(part 1 of 2)
# Autodesk Inventor assembly: Drive Roller Assembly 2
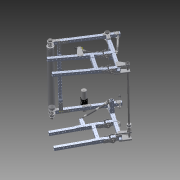
[picture p0: Inventor's stored thumbnail of the model, 180x180]
Saved by Autodesk Inventor 2014 SP1 (Build 180222100, 222)
## iProperties
Created: 2014-01-12
Part Number: Drive Roller Assembly 2
Document SubType Name: Assembly
Designer: Michael
Mass: 6489.5 g
Surface Area: 18387.5 cm^2
Volume: 1765.28 cm^3
Density: 3.67619 g/cm^3
Author: Michael
## Documents named in this file (45)
- C:\Users\Arpan\Documents\GitHub\2014buildCAD\New Collector\Drive Roller Assembly 2.iam
- C:\Users\Arpan\Documents\GitHub\2014buildCAD\Collector\Roller End Cap Drive (3-D Printed).ipt
- C:\Users\Arpan\Documents\GitHub\2014buildCAD\Collector\VersaPlanetary (Fixed).iam
- C:\Users\Arpan\Documents\GitHub\2014buildCAD\New Collector\Polycarbonate Roller 2 OD 1-16 Thick (8585K64).ipt
- C:\Users\Arpan\Documents\GitHub\2014buildCAD\New Collector\Hex Bearing 1-2 in (FR8ZZ-Hex, am-0279).ipt
- C:\Users\Arpan\Documents\GitHub\2014buildCAD\New Collector\Hex Shaft Collar 1-2 in (7552K500).ipt
- C:\Users\Arpan\Documents\GitHub\2014buildCAD\New Collector\Roller End Cap Drive (3-D Printed).ipt
- C:\Users\Arpan\Documents\GitHub\2014buildCAD\New Collector\Vex Pro End Bearing Mount.ipt
- C:\Users\Arpan\Documents\GitHub\2014buildCAD\New Collector\Vex Pro 1x1 rectangular tubing 14 in length.ipt
- C:\Users\Arpan\Documents\GitHub\2014buildCAD\New Collector\Hex Shaft Aluminum 1-2 in (am-2291).ipt
- C:\Users\Arpan\Documents\GitHub\2014buildCAD\New Collector\Timing Pulley (HTD 5mm) - 18T 9mm Double Flange, 1-2 in Hex (VexPro).ipt
- C:\Users\Arpan\Documents\GitHub\2014buildCAD\New Collector\Clamp with Piston Assembly.iam
- C:\Users\Arpan\Documents\GitHub\2014buildCAD\New Collector\Vex Pro 90 degree gusset.ipt
- C:\Users\Arpan\Documents\GitHub\2014buildCAD\New Collector\Vex Pro 1x1 rectangular tubing 2 in length.ipt
- C:\Users\Arpan\Documents\GitHub\2014buildCAD\New Collector\Hex Shaft 3-8 in (am-0855).ipt
- C:\Users\Arpan\Documents\GitHub\2014buildCAD\New Collector\Hex Shaft Collar 3-8 in (7552K300).ipt
- C:\Users\Arpan\Documents\GitHub\2014buildCAD\New Collector\Hex Shaft 1-2 in (am-0856).ipt
- C:\Users\Arpan\Documents\GitHub\2014buildCAD\New Collector\Spacer 2.ipt
- C:\Users\Arpan\Documents\GitHub\2014buildCAD\New Collector\Gusset 3 (R-R) (Custom) ipt.ipt
- C:\Users\Arpan\Documents\GitHub\2014buildCAD\New Collector\Gusset 3 (L-R) (Custom).ipt
- C:\Users\Arpan\Documents\GitHub\2014buildCAD\New Collector\Gusset 3 (L-L) (Custom) ipt.ipt
- C:\Users\Arpan\Documents\GitHub\2014buildCAD\New Collector\Gusset 3 (R-L) (Custom).ipt
- C:\Users\Arpan\Documents\GitHub\2014buildCAD\New Collector\Vex Pro 1x1 rectangular tubing 4 in length.ipt
- C:\Users\Arpan\Documents\GitHub\2014buildCAD\New Collector\Pneumatic Piston Front Flange (Lt Custom).ipt
- C:\Users\Arpan\Documents\GitHub\2014buildCAD\New Collector\Pneumatic Piston Front Flange (Rt Custom).ipt
- C:\Users\Arpan\Documents\GitHub\2014buildCAD\New Collector\Pneumatic Piston Back Flange (Rt Custom).ipt
- C:\Users\Arpan\Documents\GitHub\2014buildCAD\Duluth Collector\Bearing Mount Spacer 1-8 in.ipt
- C:\Users\Arpan\Documents\GitHub\2014buildCAD\New Collector\Vex Pro 1x1 rectangular tubing 14 in length (roller).ipt
- C:\Users\Arpan\Documents\GitHub\2014buildCAD\New Collector\Pneumatic Piston Back Flange (Right Custom).ipt
- C:\Users\Arpan\Documents\GitHub\2014buildCAD\New Collector\Hex Shaft 1-2 in 5 in long (am-0856).ipt
- C:\Users\Arpan\Documents\GitHub\2014buildCAD\New Collector\Vex Pro End Bearing Mount (Bolt).ipt
- C:\Users\Arpan\Documents\GitHub\2014buildCAD\New Collector\Bracket.ipt
- C:\Users\Arpan\Documents\GitHub\2014buildCAD\New Collector\Roller Piston 4 (.5 and 1 in Stroke, 9-16 in Bore).iam
- C:\Users\Arpan\Documents\GitHub\2014buildCAD\New Collector\Shaft Collar 3-16 in ID (6435K510).ipt
- C:\Users\Arpan\Documents\GitHub\2014buildCAD\New Collector\Standoff #8 (91125A459).ipt
- C:\Users\Arpan\Documents\GitHub\2014buildCAD\New Collector\Vex Pro 1x1 rectangular tubing 21.375 in length.ipt
- C:\Users\Arpan\Documents\GitHub\2014buildCAD\New Collector\Roller Crossbar Gusset (Custom).ipt
- C:\Users\Arpan\Documents\GitHub\2014buildCAD\New Collector\Vex Pro 1x1 rectangular tubing 2 in length (Flange Support).ipt
- C:\Users\Arpan\Documents\GitHub\2014buildCAD\New Collector\Vex Pro 90 degree gusset (1-8 in).ipt
- C:\Users\Arpan\Documents\GitHub\2014buildCAD\New Collector\Timing Pulley (HTD 5mm) - 18T 15mm 1-2 in Hex.ipt
- C:\Users\Arpan\Documents\GitHub\2014buildCAD\New Collector\Hex Spacer.ipt
- C:\Users\Arpan\Documents\GitHub\2014buildCAD\New Collector\Side Mount Custom.ipt
- C:\Users\Arpan\Documents\GitHub\2014buildCAD\New Collector\Clamp Piston ( 1 in stroke twice, 9-16 bore).iam
- C:\Users\Arpan\Documents\GitHub\2014buildCAD\New Collector\Hex Spacer 1-2 .ipt
- C:\Users\Arpan\Documents\GitHub\2014buildCAD\New Collector\Vex Pro 90 degree gusset (Special) (1-8 in).ipt
## Components (136 placed, 43 different names)
1. Roller End Cap Drive (3-D Printed):2 — Mate:154, Mate:155, Mate:1112, Flush:30, Mate:1114, Mate:1115
2. VersaPlanetary (Fixed):1 [sub-assembly] — Mate:990, Mate:991, Mate:992, Mate:1076, Mate:1077, Mate:1079, Mate:1080, Mate:1082, Mate:1083
3. Hex Bearing 1-2 in (FR8ZZ-Hex, am-0279):3 — Mate:128, Mate:129, Mate:134, Mate:797, Mate:1113
4. Roller End Cap Drive (3-D Printed):5 — Mate:1108, Mate:1109, Mate:1110
5. Hex Shaft Aluminum 1-2 in (am-2291):1 — Mate:132, Mate:133, Mate:134, Mate:154, Mate:155, Mate:172, Mate:173, Mate:179, Mate:180, Mate:467, Mate:468, Mate:797, Mate:1065, Mate:1066, Mate:1068, Mate:1069, Mate:1072, Mate:1073, Flush:30
6. Vex Pro End Bearing Mount:4 — Mate:130, Mate:131, Mate:621, Mate:798, Mate:799, Mate:873
7. Vex Pro End Bearing Mount:5 — Mate:128, Mate:129, Mate:624, Mate:800, Mate:801, Mate:866, Mate:867, Mate:868, Mate:869, Mate:870, Mate:871, Mate:872
8. Hex Bearing 1-2 in (FR8ZZ-Hex, am-0279):4 — Mate:130, Mate:131, Mate:132, Mate:133, Mate:1067
9. Hex Bearing 1-2 in (FR8ZZ-Hex, am-0279):5 — Mate:178, Mate:758, Mate:759
10. Vex Pro End Bearing Mount:7 — Mate:631, Mate:804, Mate:805
11. Vex Pro End Bearing Mount:8 — Mate:629, Mate:802, Mate:803, Mate:874, Mate:875, Mate:876, Mate:877, Mate:878, Mate:879, Mate:880, Mate:881
12. Hex Bearing 1-2 in (FR8ZZ-Hex, am-0279):6 — Mate:172, Mate:173, Mate:470, Mate:471, Mate:1111
13. Hex Shaft Collar 1-2 in (7552K500):16 — Mate:178, Mate:179, Mate:180, Flush:13
14. Clamp with Piston Assembly:1 [sub-assembly] — Mate:226, Mate:227, Flush:6, Mate:230, Mate:233, Mate:673, Mate:689, Mate:690, Mate:918, Mate:921, Mate:1104, Mate:1105, Mate:1106
15. Vex Pro 1x1 rectangular tubing 14 in length:5 — Mate:203, Mate:210, Mate:211, Mate:221, Mate:222, Mate:223, Flush:20, Mate:653, Mate:940, Mate:942, Mate:975, Mate:979, Mate:981, Mate:983, Mate:1022, Mate:1023, Flush:27, Mate:1053, Mate:1054, Mate:1055, Mate:1084, Mate:1085
16. Vex Pro 1x1 rectangular tubing 14 in length:6 — Mate:258, Mate:259, Mate:260, Mate:263, Mate:320, Mate:321, Flush:20, Mate:658, Mate:935, Mate:936, Mate:938, Mate:973, Mate:974, Mate:976, Mate:977, Mate:978, Mate:1020, Mate:1021, Flush:26, Mate:1056, Mate:1057, Mate:1058, Mate:1092
17. Vex Pro 90 degree gusset:8 — Mate:203, Mate:210, Mate:211, Mate:212, Mate:213, Mate:214
18. Vex Pro 1x1 rectangular tubing 2 in length:1 — Mate:212, Mate:213, Mate:214, Flush:25, Mate:941, Mate:961, Mate:962, Mate:964, Mate:965
19. Vex Pro 90 degree gusset:10 — Mate:221, Mate:222, Mate:223, Mate:433, Mate:434, Mate:435
20. Vex Pro 1x1 rectangular tubing 2 in length:2 — Mate:224, Mate:225, Flush:5, Mate:967, Mate:968, Mate:970, Mate:971, Mate:1086
21. Hex Shaft 3-8 in (am-0855):1 — Mate:224, Mate:225, Flush:5, Mate:226, Mate:227, Flush:6, Mate:228, Mate:229, Mate:231, Mate:232, Mate:919, Mate:920, Mate:922, Mate:923, Mate:963, Mate:966, Mate:969, Mate:972
22. Hex Shaft Collar 3-8 in (7552K300):1 — Mate:228, Mate:229, Mate:230
23. Hex Shaft Collar 3-8 in (7552K300):2 — Mate:231, Mate:232, Mate:233
24. Clamp with Piston Assembly:2 [sub-assembly] — Mate:666, Mate:668, Mate:669, Mate:916, Mate:924, Mate:1100, Mate:1101
25. Vex Pro 90 degree gusset:12 — Mate:263, Mate:320, Mate:321, Mate:324, Mate:325
26. Vex Pro 1x1 rectangular tubing 2 in length:3 — Mate:324, Mate:325, Flush:25, Mate:937, Mate:949, Mate:950, Mate:952, Mate:953
27. Vex Pro 90 degree gusset:13 — Mate:258, Mate:259, Mate:260, Mate:425, Mate:426, Mate:492
28. Vex Pro 1x1 rectangular tubing 2 in length:4 — Mate:955, Mate:956, Mate:958, Mate:959, Mate:1090, Mate:1091
29. Hex Shaft 3-8 in (am-0855):2 — Mate:915, Mate:917, Mate:925, Mate:926, Mate:951, Mate:954, Mate:957, Mate:960
30. Hex Shaft Collar 3-8 in (7552K300):3
31. Hex Shaft Collar 3-8 in (7552K300):4
32. Vex Pro 90 degree gusset:14 — Mate:476, Mate:477, Mate:478, Mate:653
33. Vex Pro 90 degree gusset:15 — Mate:650, Mate:651, Mate:652, Mate:939, Mate:1022, Mate:1023
34. Vex Pro 90 degree gusset:17 — Mate:485, Mate:486, Mate:487
35. Vex Pro 90 degree gusset:18 — Mate:656, Mate:657, Mate:658, Mate:659, Mate:1020, Mate:1021
36. Hex Shaft 1-2 in (am-0856):2 — Mate:402, Mate:403, Mate:405, Mate:406, Mate:447, Mate:448, Flush:12
37. Hex Shaft Collar 1-2 in (7552K500):18 — Mate:402, Mate:403, Mate:450, Flush:12
38. Hex Shaft Collar 1-2 in (7552K500):19 — Mate:405, Mate:406, Mate:449
39. Hex Shaft Collar 1-2 in (7552K500):21 — Mate:446, Mate:704, Mate:705, Flush:22
40. Gusset 3 (R-R) (Custom) ipt:1 — Mate:425, Mate:426, Mate:446, Mate:492, Mate:1116
41. Gusset 3 (L-R) (Custom):1 — Mate:447, Mate:448, Mate:450, Mate:461, Mate:1089, Mate:1098, Mate:1099
42. Gusset 3 (L-L) (Custom) ipt:1 — Mate:433, Mate:434, Mate:435, Mate:449
43. Gusset 3 (R-L) (Custom):1 — Mate:708, Mate:709, Mate:1034, Mate:1095, Mate:1097, Mate:1117
44. Spacer 2:3 — Mate:462, Mate:463, Mate:464, Mate:1093
45. Spacer 2:4 — Mate:458, Mate:459, Mate:460, Mate:1087, Mate:1088
46. Spacer 2:5 — Mate:458, Mate:459, Mate:460, Mate:461, Mate:1089, Mate:1099
47. Spacer 2:6 — Mate:462, Mate:463, Mate:464, Mate:1094, Mate:1095, Mate:1096, Mate:1097
48. Hex Shaft Collar 1-2 in (7552K500):22 — Mate:467, Mate:468, Mate:1112, Mate:1113
49. Hex Shaft Aluminum 1-2 in (am-2291):2 — Mate:470, Mate:471, Flush:13, Mate:633, Mate:634, Mate:758, Mate:759, Mate:1108, Mate:1109
50. Vex Pro 1x1 rectangular tubing 4 in length:1 — Mate:476, Mate:477, Mate:478, Mate:650, Mate:651, Mate:652, Mate:683, Mate:684, Mate:685
51. Vex Pro 1x1 rectangular tubing 4 in length:2 — Mate:485, Mate:486, Mate:487, Mate:656, Mate:657, Mate:659, Mate:694, Mate:699, Mate:700
52. Bearing Mount Spacer 1-8 in:1 — Mate:748, Mate:749, Mate:750, Mate:973, Mate:976
53. Bearing Mount Spacer 1-8 in:3 — Mate:743, Mate:744, Mate:745, Mate:974, Mate:978
54. Hex Bearing 1-2 in (FR8ZZ-Hex, am-0279):7 — Flush:15, Mate:560, Mate:561, Flush:23, Mate:754, Mate:755, Mate:830
55. Hex Shaft 1-2 in (am-0856):4 — Mate:560, Mate:561, Mate:562, Mate:563, Flush:23, Mate:774, Mate:829, Mate:831, Mate:833, Mate:834, Mate:1040, Mate:1043
56. Hex Bearing 1-2 in (FR8ZZ-Hex, am-0279):8 — Flush:15, Mate:746, Mate:747, Mate:774, Mate:832
57. Vex Pro 1x1 rectangular tubing 14 in length (roller):1 — Mate:562, Mate:563, Mate:621, Mate:624, Flush:21, Mate:790, Mate:791, Mate:793, Mate:798, Mate:799, Mate:800, Mate:801, Mate:862, Mate:863, Mate:864, Mate:887, Mate:903, Mate:904, Mate:909, Mate:910, Mate:912, Mate:988, Mate:989, Mate:1038, Mate:1039, Mate:1041, Mate:1042, Flush:26, Mate:1050
58. Bearing Mount Spacer 1-8 in:5 — Mate:740, Mate:741, Mate:742, Mate:983
59. Bearing Mount Spacer 1-8 in:7 — Mate:735, Mate:736, Mate:737, Mate:975, Mate:980
60. Hex Bearing 1-2 in (FR8ZZ-Hex, am-0279):9 — Flush:19, Mate:752, Mate:753, Mate:854
61. Hex Shaft 1-2 in (am-0856):5 — Flush:19, Mate:775, Mate:836, Mate:843, Mate:852, Mate:853, Mate:1046, Mate:1049
62. Hex Bearing 1-2 in (FR8ZZ-Hex, am-0279):10 — Mate:738, Mate:739, Mate:775, Mate:835
63. Vex Pro 1x1 rectangular tubing 14 in length (roller):2 — Mate:629, Mate:631, Flush:21, Mate:802, Mate:803, Mate:804, Mate:805, Mate:806, Mate:807, Mate:808, Mate:809, Mate:810, Mate:811, Mate:892, Mate:896, Mate:905, Mate:906, Mate:907, Mate:908, Mate:1044, Mate:1045, Mate:1047, Mate:1048, Flush:27
64. Hex Shaft Collar 1-2 in (7552K500):23 — Mate:633, Mate:634, Mate:1110, Mate:1111
65. Pneumatic Piston Front Flange (Rt Custom):2 — Mate:666, Mate:668, Mate:669, Mate:932, Mate:933, Mate:934, Mate:1103
66. Pneumatic Piston Front Flange (Lt Custom):1 — Mate:673, Mate:689, Mate:690, Mate:929, Mate:930, Mate:931, Mate:1107
67. Pneumatic Piston Back Flange (Rt Custom):1 — Mate:683, Mate:684, Mate:685, Mate:1028, Mate:1029, Mate:1030
68. Pneumatic Piston Back Flange (Right Custom):1 — Mate:694, Mate:699, Mate:700, Mate:1024, Mate:1025, Mate:1026
69. Hex Shaft 1-2 in 5 in long (am-0856):1 — Mate:704, Mate:705, Mate:708, Mate:709, Flush:22, Mate:946, Mate:947, Mate:1032, Mate:1033, Mate:1116
70. Vex Pro End Bearing Mount (Bolt):1 — Mate:735, Mate:736, Mate:737, Mate:738, Mate:739, Mate:979, Mate:980
71. Vex Pro End Bearing Mount (Bolt):2 — Mate:740, Mate:741, Mate:742, Mate:752, Mate:753, Mate:981
72. Vex Pro End Bearing Mount (Bolt):3 — Mate:743, Mate:744, Mate:745, Mate:746, Mate:747
73. Vex Pro End Bearing Mount (Bolt):4 — Mate:748, Mate:749, Mate:750, Mate:754, Mate:755, Mate:977
74. Bracket:1 — Mate:790, Mate:791, Mate:793, Mate:860, Mate:1059
75. Bracket:2 — Mate:806, Mate:807, Mate:808, Mate:856, Mate:1060
76. Bracket:3 — Mate:809, Mate:810, Mate:811, Mate:858
77. Hex Shaft Collar 1-2 in (7552K500):25 — Mate:829, Mate:830, Mate:831
78. Hex Shaft Collar 1-2 in (7552K500):26 — Mate:832, Mate:833, Mate:834
79. Hex Shaft Collar 1-2 in (7552K500):27 — Mate:835, Mate:836, Mate:843
80. Hex Shaft Collar 1-2 in (7552K500):29 — Mate:852, Mate:853, Mate:854
81. Shaft Collar 3-16 in ID (6435K510):1 — Mate:858, Mate:1062
82. Shaft Collar 3-16 in ID (6435K510):2 — Mate:856, Mate:1061
83. Shaft Collar 3-16 in ID (6435K510):3 — Mate:860, Mate:1063
84. Shaft Collar 3-16 in ID (6435K510):4 — Mate:865, Mate:1064
85. Bracket:4 — Mate:862, Mate:863, Mate:864, Mate:865
86. Standoff #8 (91125A459):1 — Mate:866, Mate:867
87. Standoff #8 (91125A459):2 — Mate:868, Mate:869
88. Standoff #8 (91125A459):3 — Mate:870, Mate:871
89. Standoff #8 (91125A459):4 — Mate:872, Mate:873
90. Standoff #8 (91125A459):5 — Mate:874, Mate:875
91. Standoff #8 (91125A459):6 — Mate:876, Mate:877
92. Standoff #8 (91125A459):7 — Mate:878, Mate:879
93. Standoff #8 (91125A459):8 — Mate:880, Mate:881
94. Vex Pro 1x1 rectangular tubing 21.375 in length:1 — Mate:894, Mate:897, Mate:900, Mate:901, Mate:902, Mate:911
95. Roller Crossbar Gusset (Custom):2 — Mate:887, Mate:900, Mate:901, Mate:902, Mate:903, Mate:904
96. Roller Crossbar Gusset (Custom):3 — Mate:896, Mate:897, Mate:905, Mate:906
97. Roller Crossbar Gusset (Custom):4 — Mate:892, Mate:894, Mate:907, Mate:908
98. Roller Crossbar Gusset (Custom):5 — Mate:909, Mate:910, Mate:911, Mate:912
99. Hex Shaft Collar 3-8 in (7552K300):5 — Mate:915, Mate:916, Mate:917
100. Hex Shaft Collar 3-8 in (7552K300):6 — Mate:918, Mate:919, Mate:920
101. Hex Shaft Collar 3-8 in (7552K300):7 — Mate:921, Mate:922, Mate:923
102. Hex Shaft Collar 3-8 in (7552K300):8 — Mate:924, Mate:925, Mate:926
103. Vex Pro 1x1 rectangular tubing 2 in length (Flange Support):1 — Mate:929, Mate:930, Mate:931
104. Vex Pro 1x1 rectangular tubing 2 in length (Flange Support):2 — Mate:932, Mate:933, Mate:934, Mate:1102
105. Vex Pro 90 degree gusset (1-8 in):1 — Mate:935, Mate:936, Mate:937, Mate:938
106. Vex Pro 90 degree gusset (1-8 in):2 — Mate:939, Mate:940, Mate:941, Mate:942
107. Timing Pulley (HTD 5mm) - 18T 15mm 1-2 in Hex:1 — Mate:946, Mate:947, Mate:1117
108. Hex Spacer:1 — Mate:949, Mate:950, Mate:951
109. Hex Spacer:2 — Mate:952, Mate:953, Mate:954
110. Hex Spacer:3 — Mate:955, Mate:956, Mate:957
111. Hex Spacer:4 — Mate:958, Mate:959, Mate:960
112. Hex Spacer:5 — Mate:961, Mate:962, Mate:963
113. Hex Spacer:6 — Mate:964, Mate:965, Mate:966
114. Hex Spacer:7 — Mate:967, Mate:968, Mate:969
115. Hex Spacer:8 — Mate:970, Mate:971, Mate:972
116. Side Mount Custom:1 — Mate:988, Mate:989, Mate:990, Mate:991, Mate:992, Mate:1050
117. Clamp Piston ( 1 in stroke twice, 9-16 bore):1 [sub-assembly] — Mate:1024, Mate:1025, Mate:1026, Mate:1103
118. Clamp Piston ( 1 in stroke twice, 9-16 bore):2 [sub-assembly] — Mate:1028, Mate:1029, Mate:1030, Mate:1107
119. Hex Shaft Collar 1-2 in (7552K500):30 — Mate:1032, Mate:1033, Mate:1034
120. Hex Spacer 1-2 :1 — Mate:1038, Mate:1039, Mate:1040
121. Hex Spacer 1-2 :2 — Mate:1041, Mate:1042, Mate:1043
122. Hex Spacer 1-2 :3 — Mate:1044, Mate:1045, Mate:1046
123. Hex Spacer 1-2 :4 — Mate:1047, Mate:1048, Mate:1049
124. Roller Piston 4 (.5 and 1 in Stroke, 9-16 in Bore):1 [sub-assembly] — Mate:1053, Mate:1054, Mate:1055, Mate:1060, Mate:1061, Mate:1062
125. Roller Piston 4 (.5 and 1 in Stroke, 9-16 in Bore):2 [sub-assembly] — Mate:1056, Mate:1057, Mate:1058, Mate:1059, Mate:1063, Mate:1064
126. Hex Shaft Collar 1-2 in (7552K500):31 — Mate:1065, Mate:1066, Mate:1067, Mate:1070
127. Timing Pulley (HTD 5mm) - 18T 9mm Double Flange, 1-2 in Hex (VexPro):5 — Mate:1068, Mate:1069, Mate:1070, Mate:1071
128. Hex Shaft Collar 1-2 in (7552K500):32 — Mate:1071, Mate:1072, Mate:1073, Flush:29
129. Hex Shaft Collar 1-2 in (7552K500):33 — Mate:1081, Mate:1082, Mate:1083
130. Timing Pulley (HTD 5mm) - 18T 9mm Double Flange, 1-2 in Hex (VexPro):6 — Mate:1078, Mate:1079, Mate:1080, Mate:1081
131. Hex Shaft Collar 1-2 in (7552K500):34 — Mate:1076, Flush:29, Mate:1077, Mate:1078
132. Vex Pro 90 degree gusset (1-8 in):3 — Mate:1084, Mate:1085, Mate:1086, Mate:1087, Mate:1088, Mate:1098
133. Vex Pro 90 degree gusset (1-8 in):4 — Mate:1090, Mate:1091, Mate:1092, Mate:1093, Mate:1094, Mate:1096
134. Vex Pro 90 degree gusset (Special) (1-8 in):1 — Mate:1100, Mate:1101, Mate:1102
135. Vex Pro 90 degree gusset (Special) (1-8 in):2 — Mate:1104, Mate:1105, Mate:1106
136. Polycarbonate Roller 2 OD 1-16 Thick (8585K64):1 — Mate:1114, Mate:1115
## Relationships (403: Mate 385, Flush 18)
- Mate:128: Hex Bearing 1-2 in (FR8ZZ-Hex, am-0279):3 ↔ Vex Pro End Bearing Mount:5
- Mate:129: Hex Bearing 1-2 in (FR8ZZ-Hex, am-0279):3 ↔ Vex Pro End Bearing Mount:5
- Mate:130: Vex Pro End Bearing Mount:4 ↔ Hex Bearing 1-2 in (FR8ZZ-Hex, am-0279):4
- Mate:131: Vex Pro End Bearing Mount:4 ↔ Hex Bearing 1-2 in (FR8ZZ-Hex, am-0279):4
- Mate:132: Hex Shaft Aluminum 1-2 in (am-2291):1 ↔ Hex Bearing 1-2 in (FR8ZZ-Hex, am-0279):4
- Mate:133: Hex Shaft Aluminum 1-2 in (am-2291):1 ↔ Hex Bearing 1-2 in (FR8ZZ-Hex, am-0279):4
- Mate:134: Hex Bearing 1-2 in (FR8ZZ-Hex, am-0279):3 ↔ Hex Shaft Aluminum 1-2 in (am-2291):1
- Mate:154: Roller End Cap Drive (3-D Printed):2 ↔ Hex Shaft Aluminum 1-2 in (am-2291):1
- Mate:155: Roller End Cap Drive (3-D Printed):2 ↔ Hex Shaft Aluminum 1-2 in (am-2291):1
- [Mate]: Hex Bearing 1-2 in (FR8ZZ-Hex, am-0279):5 ↔ Vex Pro End Bearing Mount:8
- [Mate]: Hex Bearing 1-2 in (FR8ZZ-Hex, am-0279):5 ↔ Vex Pro End Bearing Mount:8
- [Mate]: Vex Pro End Bearing Mount:7 ↔ Hex Bearing 1-2 in (FR8ZZ-Hex, am-0279):6
- [Mate]: Vex Pro End Bearing Mount:7 ↔ Hex Bearing 1-2 in (FR8ZZ-Hex, am-0279):6
- Mate:172: Hex Shaft Aluminum 1-2 in (am-2291):1 ↔ Hex Bearing 1-2 in (FR8ZZ-Hex, am-0279):6
- Mate:173: Hex Shaft Aluminum 1-2 in (am-2291):1 ↔ Hex Bearing 1-2 in (FR8ZZ-Hex, am-0279):6
- Mate:178: Hex Bearing 1-2 in (FR8ZZ-Hex, am-0279):5 ↔ Hex Shaft Collar 1-2 in (7552K500):16
- Mate:179: Hex Shaft Aluminum 1-2 in (am-2291):1 ↔ Hex Shaft Collar 1-2 in (7552K500):16
- Mate:180: Hex Shaft Aluminum 1-2 in (am-2291):1 ↔ Hex Shaft Collar 1-2 in (7552K500):16
- Mate:203: Vex Pro 1x1 rectangular tubing 14 in length:5 ↔ Vex Pro 90 degree gusset:8
- Mate:210: Vex Pro 1x1 rectangular tubing 14 in length:5 ↔ Vex Pro 90 degree gusset:8
- Mate:211: Vex Pro 1x1 rectangular tubing 14 in length:5 ↔ Vex Pro 90 degree gusset:8
- Mate:212: Vex Pro 90 degree gusset:8 ↔ Vex Pro 1x1 rectangular tubing 2 in length:1
- Mate:213: Vex Pro 90 degree gusset:8 ↔ Vex Pro 1x1 rectangular tubing 2 in length:1
- Mate:214: Vex Pro 90 degree gusset:8 ↔ Vex Pro 1x1 rectangular tubing 2 in length:1
- [Mate]: Vex Pro 90 degree gusset:10 ↔ Vex Pro 1x1 rectangular tubing 2 in length:2
- [Mate]: Vex Pro 90 degree gusset:10 ↔ Vex Pro 1x1 rectangular tubing 2 in length:2
- [Mate]: Vex Pro 90 degree gusset:10 ↔ Vex Pro 1x1 rectangular tubing 2 in length:2
- Mate:221: Vex Pro 1x1 rectangular tubing 14 in length:5 ↔ Vex Pro 90 degree gusset:10
- Mate:222: Vex Pro 1x1 rectangular tubing 14 in length:5 ↔ Vex Pro 90 degree gusset:10
- Mate:223: Vex Pro 1x1 rectangular tubing 14 in length:5 ↔ Vex Pro 90 degree gusset:10
- Mate:224: Vex Pro 1x1 rectangular tubing 2 in length:2 ↔ Hex Shaft 3-8 in (am-0855):1
- Mate:225: Vex Pro 1x1 rectangular tubing 2 in length:2 ↔ Hex Shaft 3-8 in (am-0855):1
- Flush:5 (-19.05 mm): Vex Pro 1x1 rectangular tubing 2 in length:2 ↔ Hex Shaft 3-8 in (am-0855):1
- Mate:226: Clamp with Piston Assembly:1 ↔ Hex Shaft 3-8 in (am-0855):1
- Mate:227: Clamp with Piston Assembly:1 ↔ Hex Shaft 3-8 in (am-0855):1
- Flush:6 (-7.1437 mm): Clamp with Piston Assembly:1 ↔ Hex Shaft 3-8 in (am-0855):1
- Mate:228: Hex Shaft 3-8 in (am-0855):1 ↔ Hex Shaft Collar 3-8 in (7552K300):1
- Mate:229: Hex Shaft 3-8 in (am-0855):1 ↔ Hex Shaft Collar 3-8 in (7552K300):1
- Mate:230: Clamp with Piston Assembly:1 ↔ Hex Shaft Collar 3-8 in (7552K300):1
- Mate:231: Hex Shaft 3-8 in (am-0855):1 ↔ Hex Shaft Collar 3-8 in (7552K300):2
- Mate:232: Hex Shaft 3-8 in (am-0855):1 ↔ Hex Shaft Collar 3-8 in (7552K300):2
- Mate:233: Clamp with Piston Assembly:1 ↔ Hex Shaft Collar 3-8 in (7552K300):2
- [Mate]: Vex Pro 90 degree gusset:12 ↔ Vex Pro 1x1 rectangular tubing 2 in length:3
- [Mate]: Vex Pro 90 degree gusset:13 ↔ Vex Pro 1x1 rectangular tubing 2 in length:4
- [Mate]: Vex Pro 90 degree gusset:13 ↔ Vex Pro 1x1 rectangular tubing 2 in length:4
- [Mate]: Vex Pro 90 degree gusset:13 ↔ Vex Pro 1x1 rectangular tubing 2 in length:4
- [Mate]: Vex Pro 1x1 rectangular tubing 2 in length:4 ↔ Hex Shaft 3-8 in (am-0855):2
- [Mate]: Vex Pro 1x1 rectangular tubing 2 in length:4 ↔ Hex Shaft 3-8 in (am-0855):2
- [Flush] (-19.05 mm): Vex Pro 1x1 rectangular tubing 2 in length:4 ↔ Hex Shaft 3-8 in (am-0855):2
- [Mate]: Clamp with Piston Assembly:2 ↔ Hex Shaft 3-8 in (am-0855):2
- [Mate]: Clamp with Piston Assembly:2 ↔ Hex Shaft 3-8 in (am-0855):2
- [Flush] (-7.1437 mm): Clamp with Piston Assembly:2 ↔ Hex Shaft 3-8 in (am-0855):2
- [Mate]: Hex Shaft 3-8 in (am-0855):2 ↔ Hex Shaft Collar 3-8 in (7552K300):3
- [Mate]: Hex Shaft 3-8 in (am-0855):2 ↔ Hex Shaft Collar 3-8 in (7552K300):3
- [Mate]: Clamp with Piston Assembly:2 ↔ Hex Shaft Collar 3-8 in (7552K300):3
- [Mate]: Hex Shaft 3-8 in (am-0855):2 ↔ Hex Shaft Collar 3-8 in (7552K300):4
- [Mate]: Hex Shaft 3-8 in (am-0855):2 ↔ Hex Shaft Collar 3-8 in (7552K300):4
- [Mate]: Clamp with Piston Assembly:2 ↔ Hex Shaft Collar 3-8 in (7552K300):4
- Mate:258: Vex Pro 1x1 rectangular tubing 14 in length:6 ↔ Vex Pro 90 degree gusset:13
- Mate:259: Vex Pro 1x1 rectangular tubing 14 in length:6 ↔ Vex Pro 90 degree gusset:13
- Mate:260: Vex Pro 1x1 rectangular tubing 14 in length:6 ↔ Vex Pro 90 degree gusset:13
- Mate:263: Vex Pro 1x1 rectangular tubing 14 in length:6 ↔ Vex Pro 90 degree gusset:12
- Mate:320: Vex Pro 1x1 rectangular tubing 14 in length:6 ↔ Vex Pro 90 degree gusset:12
- Mate:321: Vex Pro 1x1 rectangular tubing 14 in length:6 ↔ Vex Pro 90 degree gusset:12
- Mate:324: Vex Pro 90 degree gusset:12 ↔ Vex Pro 1x1 rectangular tubing 2 in length:3
- Mate:325: Vex Pro 90 degree gusset:12 ↔ Vex Pro 1x1 rectangular tubing 2 in length:3
- Mate:402: Hex Shaft 1-2 in (am-0856):2 ↔ Hex Shaft Collar 1-2 in (7552K500):18
- Mate:403: Hex Shaft 1-2 in (am-0856):2 ↔ Hex Shaft Collar 1-2 in (7552K500):18
- Mate:405: Hex Shaft 1-2 in (am-0856):2 ↔ Hex Shaft Collar 1-2 in (7552K500):19
- Mate:406: Hex Shaft 1-2 in (am-0856):2 ↔ Hex Shaft Collar 1-2 in (7552K500):19
- Mate:425: Vex Pro 90 degree gusset:13 ↔ Gusset 3 (R-R) (Custom) ipt:1
- Mate:426: Vex Pro 90 degree gusset:13 ↔ Gusset 3 (R-R) (Custom) ipt:1
- Mate:433: Vex Pro 90 degree gusset:10 ↔ Gusset 3 (L-L) (Custom) ipt:1
- Mate:434: Vex Pro 90 degree gusset:10 ↔ Gusset 3 (L-L) (Custom) ipt:1
- Mate:435: Vex Pro 90 degree gusset:10 ↔ Gusset 3 (L-L) (Custom) ipt:1
- Mate:446: Hex Shaft Collar 1-2 in (7552K500):21 ↔ Gusset 3 (R-R) (Custom) ipt:1
- Mate:447: Hex Shaft 1-2 in (am-0856):2 ↔ Gusset 3 (L-R) (Custom):1
- Mate:448: Hex Shaft 1-2 in (am-0856):2 ↔ Gusset 3 (L-R) (Custom):1
- Mate:449: Hex Shaft Collar 1-2 in (7552K500):19 ↔ Gusset 3 (L-L) (Custom) ipt:1
- Mate:450: Hex Shaft Collar 1-2 in (7552K500):18 ↔ Gusset 3 (L-R) (Custom):1
- Mate:458: Spacer 2:4 ↔ Spacer 2:5
- Mate:459: Spacer 2:4 ↔ Spacer 2:5
- Mate:460: Spacer 2:4 ↔ Spacer 2:5
- Mate:461: Gusset 3 (L-R) (Custom):1 ↔ Spacer 2:5
- Mate:462: Spacer 2:3 ↔ Spacer 2:6
- Mate:463: Spacer 2:3 ↔ Spacer 2:6
- Mate:464: Spacer 2:3 ↔ Spacer 2:6
- Flush:12 (-9.525 mm): Hex Shaft 1-2 in (am-0856):2 ↔ Hex Shaft Collar 1-2 in (7552K500):18
- Mate:467: Hex Shaft Aluminum 1-2 in (am-2291):1 ↔ Hex Shaft Collar 1-2 in (7552K500):22
- Mate:468: Hex Shaft Aluminum 1-2 in (am-2291):1 ↔ Hex Shaft Collar 1-2 in (7552K500):22
- Mate:470: Hex Bearing 1-2 in (FR8ZZ-Hex, am-0279):6 ↔ Hex Shaft Aluminum 1-2 in (am-2291):2
- Mate:471: Hex Bearing 1-2 in (FR8ZZ-Hex, am-0279):6 ↔ Hex Shaft Aluminum 1-2 in (am-2291):2
- Flush:13 (-3.175 mm): Hex Shaft Collar 1-2 in (7552K500):16 ↔ Hex Shaft Aluminum 1-2 in (am-2291):2
- Mate:476: Vex Pro 90 degree gusset:14 ↔ Vex Pro 1x1 rectangular tubing 4 in length:1
- Mate:477: Vex Pro 90 degree gusset:14 ↔ Vex Pro 1x1 rectangular tubing 4 in length:1
- Mate:478: Vex Pro 90 degree gusset:14 ↔ Vex Pro 1x1 rectangular tubing 4 in length:1
- Mate:485: Vex Pro 90 degree gusset:17 ↔ Vex Pro 1x1 rectangular tubing 4 in length:2
- Mate:486: Vex Pro 90 degree gusset:17 ↔ Vex Pro 1x1 rectangular tubing 4 in length:2
- Mate:487: Vex Pro 90 degree gusset:17 ↔ Vex Pro 1x1 rectangular tubing 4 in length:2
- Mate:492: Vex Pro 90 degree gusset:13 ↔ Gusset 3 (R-R) (Custom) ipt:1
- Flush:15: Hex Bearing 1-2 in (FR8ZZ-Hex, am-0279):7 ↔ Hex Bearing 1-2 in (FR8ZZ-Hex, am-0279):8
- Mate:560: Hex Bearing 1-2 in (FR8ZZ-Hex, am-0279):7 ↔ Hex Shaft 1-2 in (am-0856):4
- Mate:561: Hex Bearing 1-2 in (FR8ZZ-Hex, am-0279):7 ↔ Hex Shaft 1-2 in (am-0856):4
- Mate:562: Hex Shaft 1-2 in (am-0856):4 ↔ Vex Pro 1x1 rectangular tubing 14 in length (roller):1
- Mate:563: Hex Shaft 1-2 in (am-0856):4 ↔ Vex Pro 1x1 rectangular tubing 14 in length (roller):1
- [Flush]: Hex Bearing 1-2 in (FR8ZZ-Hex, am-0279):9 ↔ Hex Bearing 1-2 in (FR8ZZ-Hex, am-0279):10
- [Mate]: Hex Bearing 1-2 in (FR8ZZ-Hex, am-0279):9 ↔ Hex Shaft 1-2 in (am-0856):5
- [Mate]: Hex Bearing 1-2 in (FR8ZZ-Hex, am-0279):9 ↔ Hex Shaft 1-2 in (am-0856):5
- [Mate]: Hex Shaft 1-2 in (am-0856):5 ↔ Vex Pro 1x1 rectangular tubing 14 in length (roller):2
- [Mate]: Hex Shaft 1-2 in (am-0856):5 ↔ Vex Pro 1x1 rectangular tubing 14 in length (roller):2
- Flush:19 (15.0812 mm): Hex Bearing 1-2 in (FR8ZZ-Hex, am-0279):9 ↔ Hex Shaft 1-2 in (am-0856):5
- Mate:621: Vex Pro End Bearing Mount:4 ↔ Vex Pro 1x1 rectangular tubing 14 in length (roller):1
- Mate:624: Vex Pro End Bearing Mount:5 ↔ Vex Pro 1x1 rectangular tubing 14 in length (roller):1
- Mate:629: Vex Pro End Bearing Mount:8 ↔ Vex Pro 1x1 rectangular tubing 14 in length (roller):2
- Flush:20: Vex Pro 1x1 rectangular tubing 14 in length:5 ↔ Vex Pro 1x1 rectangular tubing 14 in length:6
- Mate:631: Vex Pro End Bearing Mount:7 ↔ Vex Pro 1x1 rectangular tubing 14 in length (roller):2
- Mate:633: Hex Shaft Aluminum 1-2 in (am-2291):2 ↔ Hex Shaft Collar 1-2 in (7552K500):23
- Mate:634: Hex Shaft Aluminum 1-2 in (am-2291):2 ↔ Hex Shaft Collar 1-2 in (7552K500):23
- Flush:21: Vex Pro 1x1 rectangular tubing 14 in length (roller):1 ↔ Vex Pro 1x1 rectangular tubing 14 in length (roller):2
- Mate:650: Vex Pro 90 degree gusset:15 ↔ Vex Pro 1x1 rectangular tubing 4 in length:1
- Mate:651: Vex Pro 90 degree gusset:15 ↔ Vex Pro 1x1 rectangular tubing 4 in length:1
- Mate:652: Vex Pro 90 degree gusset:15 ↔ Vex Pro 1x1 rectangular tubing 4 in length:1
- Mate:653: Vex Pro 1x1 rectangular tubing 14 in length:5 ↔ Vex Pro 90 degree gusset:14
- Mate:656: Vex Pro 90 degree gusset:18 ↔ Vex Pro 1x1 rectangular tubing 4 in length:2
- Mate:657: Vex Pro 90 degree gusset:18 ↔ Vex Pro 1x1 rectangular tubing 4 in length:2
- Mate:658: Vex Pro 1x1 rectangular tubing 14 in length:6 ↔ Vex Pro 90 degree gusset:18
- Mate:659: Vex Pro 90 degree gusset:18 ↔ Vex Pro 1x1 rectangular tubing 4 in length:2
- Mate:666: Clamp with Piston Assembly:2 ↔ Pneumatic Piston Front Flange (Rt Custom):2
- Mate:668: Clamp with Piston Assembly:2 ↔ Pneumatic Piston Front Flange (Rt Custom):2
- Mate:669: Clamp with Piston Assembly:2 ↔ Pneumatic Piston Front Flange (Rt Custom):2
- Mate:673: Clamp with Piston Assembly:1 ↔ Pneumatic Piston Front Flange (Lt Custom):1
- Mate:683: Vex Pro 1x1 rectangular tubing 4 in length:1 ↔ Pneumatic Piston Back Flange (Rt Custom):1
- Mate:684: Vex Pro 1x1 rectangular tubing 4 in length:1 ↔ Pneumatic Piston Back Flange (Rt Custom):1
- Mate:685: Vex Pro 1x1 rectangular tubing 4 in length:1 ↔ Pneumatic Piston Back Flange (Rt Custom):1
- Mate:689: Clamp with Piston Assembly:1 ↔ Pneumatic Piston Front Flange (Lt Custom):1
- Mate:690: Clamp with Piston Assembly:1 ↔ Pneumatic Piston Front Flange (Lt Custom):1
- Mate:694: Vex Pro 1x1 rectangular tubing 4 in length:2 ↔ Pneumatic Piston Back Flange (Right Custom):1
- Mate:699: Vex Pro 1x1 rectangular tubing 4 in length:2 ↔ Pneumatic Piston Back Flange (Right Custom):1
- Mate:700: Vex Pro 1x1 rectangular tubing 4 in length:2 ↔ Pneumatic Piston Back Flange (Right Custom):1
- Mate:704: Hex Shaft Collar 1-2 in (7552K500):21 ↔ Hex Shaft 1-2 in 5 in long (am-0856):1
- Mate:705: Hex Shaft Collar 1-2 in (7552K500):21 ↔ Hex Shaft 1-2 in 5 in long (am-0856):1
- Mate:708: Gusset 3 (R-L) (Custom):1 ↔ Hex Shaft 1-2 in 5 in long (am-0856):1
- Mate:709: Gusset 3 (R-L) (Custom):1 ↔ Hex Shaft 1-2 in 5 in long (am-0856):1
- Flush:22 (-3.175 mm): Hex Shaft Collar 1-2 in (7552K500):21 ↔ Hex Shaft 1-2 in 5 in long (am-0856):1
- Mate:735: Bearing Mount Spacer 1-8 in:7 ↔ Vex Pro End Bearing Mount (Bolt):1
- Mate:736: Bearing Mount Spacer 1-8 in:7 ↔ Vex Pro End Bearing Mount (Bolt):1
- Mate:737: Bearing Mount Spacer 1-8 in:7 ↔ Vex Pro End Bearing Mount (Bolt):1
- Mate:738: Hex Bearing 1-2 in (FR8ZZ-Hex, am-0279):10 ↔ Vex Pro End Bearing Mount (Bolt):1
- Mate:739: Hex Bearing 1-2 in (FR8ZZ-Hex, am-0279):10 ↔ Vex Pro End Bearing Mount (Bolt):1
- Mate:740: Bearing Mount Spacer 1-8 in:5 ↔ Vex Pro End Bearing Mount (Bolt):2
- Mate:741: Bearing Mount Spacer 1-8 in:5 ↔ Vex Pro End Bearing Mount (Bolt):2
- Mate:742: Bearing Mount Spacer 1-8 in:5 ↔ Vex Pro End Bearing Mount (Bolt):2
- Flush:23 (-9.525 mm): Hex Bearing 1-2 in (FR8ZZ-Hex, am-0279):7 ↔ Hex Shaft 1-2 in (am-0856):4
- Mate:743: Bearing Mount Spacer 1-8 in:3 ↔ Vex Pro End Bearing Mount (Bolt):3
- Mate:744: Bearing Mount Spacer 1-8 in:3 ↔ Vex Pro End Bearing Mount (Bolt):3
- Mate:745: Bearing Mount Spacer 1-8 in:3 ↔ Vex Pro End Bearing Mount (Bolt):3
- Mate:746: Hex Bearing 1-2 in (FR8ZZ-Hex, am-0279):8 ↔ Vex Pro End Bearing Mount (Bolt):3
- Mate:747: Hex Bearing 1-2 in (FR8ZZ-Hex, am-0279):8 ↔ Vex Pro End Bearing Mount (Bolt):3
- Mate:748: Bearing Mount Spacer 1-8 in:1 ↔ Vex Pro End Bearing Mount (Bolt):4
- Mate:749: Bearing Mount Spacer 1-8 in:1 ↔ Vex Pro End Bearing Mount (Bolt):4
- Mate:750: Bearing Mount Spacer 1-8 in:1 ↔ Vex Pro End Bearing Mount (Bolt):4
- Mate:752: Hex Bearing 1-2 in (FR8ZZ-Hex, am-0279):9 ↔ Vex Pro End Bearing Mount (Bolt):2
- Mate:753: Hex Bearing 1-2 in (FR8ZZ-Hex, am-0279):9 ↔ Vex Pro End Bearing Mount (Bolt):2
- Mate:754: Hex Bearing 1-2 in (FR8ZZ-Hex, am-0279):7 ↔ Vex Pro End Bearing Mount (Bolt):4
- Mate:755: Hex Bearing 1-2 in (FR8ZZ-Hex, am-0279):7 ↔ Vex Pro End Bearing Mount (Bolt):4
- Mate:758: Hex Bearing 1-2 in (FR8ZZ-Hex, am-0279):5 ↔ Hex Shaft Aluminum 1-2 in (am-2291):2
- Mate:759: Hex Bearing 1-2 in (FR8ZZ-Hex, am-0279):5 ↔ Hex Shaft Aluminum 1-2 in (am-2291):2
- Mate:774: Hex Shaft 1-2 in (am-0856):4 ↔ Hex Bearing 1-2 in (FR8ZZ-Hex, am-0279):8
- Mate:775: Hex Shaft 1-2 in (am-0856):5 ↔ Hex Bearing 1-2 in (FR8ZZ-Hex, am-0279):10
- Mate:790: Vex Pro 1x1 rectangular tubing 14 in length (roller):1 ↔ Bracket:1
- Mate:791: Vex Pro 1x1 rectangular tubing 14 in length (roller):1 ↔ Bracket:1
- Mate:793: Vex Pro 1x1 rectangular tubing 14 in length (roller):1 ↔ Bracket:1
- Mate:797: Hex Bearing 1-2 in (FR8ZZ-Hex, am-0279):3 ↔ Hex Shaft Aluminum 1-2 in (am-2291):1
- Mate:798: Vex Pro End Bearing Mount:4 ↔ Vex Pro 1x1 rectangular tubing 14 in length (roller):1
- Mate:799: Vex Pro End Bearing Mount:4 ↔ Vex Pro 1x1 rectangular tubing 14 in length (roller):1
- Mate:800: Vex Pro End Bearing Mount:5 ↔ Vex Pro 1x1 rectangular tubing 14 in length (roller):1
- Mate:801: Vex Pro End Bearing Mount:5 ↔ Vex Pro 1x1 rectangular tubing 14 in length (roller):1
- Mate:802: Vex Pro End Bearing Mount:8 ↔ Vex Pro 1x1 rectangular tubing 14 in length (roller):2
- Mate:803: Vex Pro End Bearing Mount:8 ↔ Vex Pro 1x1 rectangular tubing 14 in length (roller):2
- Mate:804: Vex Pro End Bearing Mount:7 ↔ Vex Pro 1x1 rectangular tubing 14 in length (roller):2
- Mate:805: Vex Pro End Bearing Mount:7 ↔ Vex Pro 1x1 rectangular tubing 14 in length (roller):2
- Mate:806: Vex Pro 1x1 rectangular tubing 14 in length (roller):2 ↔ Bracket:2
- Mate:807: Vex Pro 1x1 rectangular tubing 14 in length (roller):2 ↔ Bracket:2
- Mate:808: Vex Pro 1x1 rectangular tubing 14 in length (roller):2 ↔ Bracket:2
- Mate:809: Vex Pro 1x1 rectangular tubing 14 in length (roller):2 ↔ Bracket:3
- Mate:810: Vex Pro 1x1 rectangular tubing 14 in length (roller):2 ↔ Bracket:3
- Mate:811: Vex Pro 1x1 rectangular tubing 14 in length (roller):2 ↔ Bracket:3
- Flush:25: Vex Pro 1x1 rectangular tubing 2 in length:1 ↔ Vex Pro 1x1 rectangular tubing 2 in length:3
- Mate:829: Hex Shaft 1-2 in (am-0856):4 ↔ Hex Shaft Collar 1-2 in (7552K500):25
- Mate:830: Hex Bearing 1-2 in (FR8ZZ-Hex, am-0279):7 ↔ Hex Shaft Collar 1-2 in (7552K500):25
- Mate:831: Hex Shaft 1-2 in (am-0856):4 ↔ Hex Shaft Collar 1-2 in (7552K500):25
- Mate:832: Hex Bearing 1-2 in (FR8ZZ-Hex, am-0279):8 ↔ Hex Shaft Collar 1-2 in (7552K500):26
- Mate:833: Hex Shaft 1-2 in (am-0856):4 ↔ Hex Shaft Collar 1-2 in (7552K500):26
- Mate:834: Hex Shaft 1-2 in (am-0856):4 ↔ Hex Shaft Collar 1-2 in (7552K500):26
- Mate:835: Hex Bearing 1-2 in (FR8ZZ-Hex, am-0279):10 ↔ Hex Shaft Collar 1-2 in (7552K500):27
- Mate:836: Hex Shaft 1-2 in (am-0856):5 ↔ Hex Shaft Collar 1-2 in (7552K500):27
- Mate:843: Hex Shaft 1-2 in (am-0856):5 ↔ Hex Shaft Collar 1-2 in (7552K500):27
- Mate:852: Hex Shaft 1-2 in (am-0856):5 ↔ Hex Shaft Collar 1-2 in (7552K500):29
- Mate:853: Hex Shaft 1-2 in (am-0856):5 ↔ Hex Shaft Collar 1-2 in (7552K500):29
- Mate:854: Hex Bearing 1-2 in (FR8ZZ-Hex, am-0279):9 ↔ Hex Shaft Collar 1-2 in (7552K500):29
- Mate:856: Bracket:2 ↔ Shaft Collar 3-16 in ID (6435K510):2
- Mate:858: Bracket:3 ↔ Shaft Collar 3-16 in ID (6435K510):1
- Mate:860: Bracket:1 ↔ Shaft Collar 3-16 in ID (6435K510):3
- Mate:862: Vex Pro 1x1 rectangular tubing 14 in length (roller):1 ↔ Bracket:4
- Mate:863: Vex Pro 1x1 rectangular tubing 14 in length (roller):1 ↔ Bracket:4
- Mate:864: Vex Pro 1x1 rectangular tubing 14 in length (roller):1 ↔ Bracket:4
- Mate:865: Shaft Collar 3-16 in ID (6435K510):4 ↔ Bracket:4
- Mate:866: Vex Pro End Bearing Mount:5 ↔ Standoff #8 (91125A459):1
- Mate:867: Vex Pro End Bearing Mount:5 ↔ Standoff #8 (91125A459):1
- Mate:868: Vex Pro End Bearing Mount:5 ↔ Standoff #8 (91125A459):2
- Mate:869: Vex Pro End Bearing Mount:5 ↔ Standoff #8 (91125A459):2
- Mate:870: Vex Pro End Bearing Mount:5 ↔ Standoff #8 (91125A459):3
- Mate:871: Vex Pro End Bearing Mount:5 ↔ Standoff #8 (91125A459):3
- Mate:872: Vex Pro End Bearing Mount:5 ↔ Standoff #8 (91125A459):4
- Mate:873: Vex Pro End Bearing Mount:4 ↔ Standoff #8 (91125A459):4
- Mate:874: Vex Pro End Bearing Mount:8 ↔ Standoff #8 (91125A459):5
- Mate:875: Vex Pro End Bearing Mount:8 ↔ Standoff #8 (91125A459):5
- Mate:876: Vex Pro End Bearing Mount:8 ↔ Standoff #8 (91125A459):6
- Mate:877: Vex Pro End Bearing Mount:8 ↔ Standoff #8 (91125A459):6
- Mate:878: Vex Pro End Bearing Mount:8 ↔ Standoff #8 (91125A459):7
- Mate:879: Vex Pro End Bearing Mount:8 ↔ Standoff #8 (91125A459):7
- Mate:880: Vex Pro End Bearing Mount:8 ↔ Standoff #8 (91125A459):8
- Mate:881: Vex Pro End Bearing Mount:8 ↔ Standoff #8 (91125A459):8
- Mate:887: Vex Pro 1x1 rectangular tubing 14 in length (roller):1 ↔ Roller Crossbar Gusset (Custom):2
- Mate:892: Vex Pro 1x1 rectangular tubing 14 in length (roller):2 ↔ Roller Crossbar Gusset (Custom):4
- Mate:894: Vex Pro 1x1 rectangular tubing 21.375 in length:1 ↔ Roller Crossbar Gusset (Custom):4
- Mate:896: Vex Pro 1x1 rectangular tubing 14 in length (roller):2 ↔ Roller Crossbar Gusset (Custom):3
- Mate:897: Vex Pro 1x1 rectangular tubing 21.375 in length:1 ↔ Roller Crossbar Gusset (Custom):3
- Mate:900: Vex Pro 1x1 rectangular tubing 21.375 in length:1 ↔ Roller Crossbar Gusset (Custom):2
- Mate:901: Vex Pro 1x1 rectangular tubing 21.375 in length:1 ↔ Roller Crossbar Gusset (Custom):2
- Mate:902: Vex Pro 1x1 rectangular tubing 21.375 in length:1 ↔ Roller Crossbar Gusset (Custom):2
- Mate:903: Vex Pro 1x1 rectangular tubing 14 in length (roller):1 ↔ Roller Crossbar Gusset (Custom):2
- Mate:904: Vex Pro 1x1 rectangular tubing 14 in length (roller):1 ↔ Roller Crossbar Gusset (Custom):2
- Mate:905: Vex Pro 1x1 rectangular tubing 14 in length (roller):2 ↔ Roller Crossbar Gusset (Custom):3
- Mate:906: Vex Pro 1x1 rectangular tubing 14 in length (roller):2 ↔ Roller Crossbar Gusset (Custom):3
- Mate:907: Vex Pro 1x1 rectangular tubing 14 in length (roller):2 ↔ Roller Crossbar Gusset (Custom):4
- Mate:908: Vex Pro 1x1 rectangular tubing 14 in length (roller):2 ↔ Roller Crossbar Gusset (Custom):4
- Mate:909: Vex Pro 1x1 rectangular tubing 14 in length (roller):1 ↔ Roller Crossbar Gusset (Custom):5
- Mate:910: Vex Pro 1x1 rectangular tubing 14 in length (roller):1 ↔ Roller Crossbar Gusset (Custom):5
- Mate:911: Vex Pro 1x1 rectangular tubing 21.375 in length:1 ↔ Roller Crossbar Gusset (Custom):5
- Mate:912: Vex Pro 1x1 rectangular tubing 14 in length (roller):1 ↔ Roller Crossbar Gusset (Custom):5
- Mate:915: Hex Shaft 3-8 in (am-0855):2 ↔ Hex Shaft Collar 3-8 in (7552K300):5
- Mate:916: Clamp with Piston Assembly:2 ↔ Hex Shaft Collar 3-8 in (7552K300):5
- Mate:917: Hex Shaft 3-8 in (am-0855):2 ↔ Hex Shaft Collar 3-8 in (7552K300):5
- Mate:918: Clamp with Piston Assembly:1 ↔ Hex Shaft Collar 3-8 in (7552K300):6
- Mate:919: Hex Shaft 3-8 in (am-0855):1 ↔ Hex Shaft Collar 3-8 in (7552K300):6
- Mate:920: Hex Shaft 3-8 in (am-0855):1 ↔ Hex Shaft Collar 3-8 in (7552K300):6
- Mate:921: Clamp with Piston Assembly:1 ↔ Hex Shaft Collar 3-8 in (7552K300):7
- Mate:922: Hex Shaft 3-8 in (am-0855):1 ↔ Hex Shaft Collar 3-8 in (7552K300):7
- Mate:923: Hex Shaft 3-8 in (am-0855):1 ↔ Hex Shaft Collar 3-8 in (7552K300):7
- Mate:924: Clamp with Piston Assembly:2 ↔ Hex Shaft Collar 3-8 in (7552K300):8
- Mate:925: Hex Shaft 3-8 in (am-0855):2 ↔ Hex Shaft Collar 3-8 in (7552K300):8
- Mate:926: Hex Shaft 3-8 in (am-0855):2 ↔ Hex Shaft Collar 3-8 in (7552K300):8
- Mate:929: Pneumatic Piston Front Flange (Lt Custom):1 ↔ Vex Pro 1x1 rectangular tubing 2 in length (Flange Support):1
- Mate:930: Pneumatic Piston Front Flange (Lt Custom):1 ↔ Vex Pro 1x1 rectangular tubing 2 in length (Flange Support):1
- Mate:931: Pneumatic Piston Front Flange (Lt Custom):1 ↔ Vex Pro 1x1 rectangular tubing 2 in length (Flange Support):1
- Mate:932: Pneumatic Piston Front Flange (Rt Custom):2 ↔ Vex Pro 1x1 rectangular tubing 2 in length (Flange Support):2
- Mate:933: Pneumatic Piston Front Flange (Rt Custom):2 ↔ Vex Pro 1x1 rectangular tubing 2 in length (Flange Support):2
- Mate:934: Pneumatic Piston Front Flange (Rt Custom):2 ↔ Vex Pro 1x1 rectangular tubing 2 in length (Flange Support):2
- Mate:935: Vex Pro 1x1 rectangular tubing 14 in length:6 ↔ Vex Pro 90 degree gusset (1-8 in):1
- Mate:936: Vex Pro 1x1 rectangular tubing 14 in length:6 ↔ Vex Pro 90 degree gusset (1-8 in):1
- Mate:937: Vex Pro 1x1 rectangular tubing 2 in length:3 ↔ Vex Pro 90 degree gusset (1-8 in):1
- Mate:938: Vex Pro 1x1 rectangular tubing 14 in length:6 ↔ Vex Pro 90 degree gusset (1-8 in):1
- Mate:939: Vex Pro 90 degree gusset:15 ↔ Vex Pro 90 degree gusset (1-8 in):2
- Mate:940: Vex Pro 1x1 rectangular tubing 14 in length:5 ↔ Vex Pro 90 degree gusset (1-8 in):2
- Mate:941: Vex Pro 1x1 rectangular tubing 2 in length:1 ↔ Vex Pro 90 degree gusset (1-8 in):2
- Mate:942: Vex Pro 1x1 rectangular tubing 14 in length:5 ↔ Vex Pro 90 degree gusset (1-8 in):2
- Mate:946: Hex Shaft 1-2 in 5 in long (am-0856):1 ↔ Timing Pulley (HTD 5mm) - 18T 15mm 1-2 in Hex:1
- Mate:947: Hex Shaft 1-2 in 5 in long (am-0856):1 ↔ Timing Pulley (HTD 5mm) - 18T 15mm 1-2 in Hex:1
- Mate:949: Vex Pro 1x1 rectangular tubing 2 in length:3 ↔ Hex Spacer:1
- Mate:950: Vex Pro 1x1 rectangular tubing 2 in length:3 ↔ Hex Spacer:1
- Mate:951: Hex Shaft 3-8 in (am-0855):2 ↔ Hex Spacer:1
- Mate:952: Vex Pro 1x1 rectangular tubing 2 in length:3 ↔ Hex Spacer:2
- Mate:953: Vex Pro 1x1 rectangular tubing 2 in length:3 ↔ Hex Spacer:2
- Mate:954: Hex Shaft 3-8 in (am-0855):2 ↔ Hex Spacer:2
- Mate:955: Vex Pro 1x1 rectangular tubing 2 in length:4 ↔ Hex Spacer:3
- Mate:956: Vex Pro 1x1 rectangular tubing 2 in length:4 ↔ Hex Spacer:3
- Mate:957: Hex Shaft 3-8 in (am-0855):2 ↔ Hex Spacer:3
- Mate:958: Vex Pro 1x1 rectangular tubing 2 in length:4 ↔ Hex Spacer:4
- Mate:959: Vex Pro 1x1 rectangular tubing 2 in length:4 ↔ Hex Spacer:4
- Mate:960: Hex Shaft 3-8 in (am-0855):2 ↔ Hex Spacer:4
- Mate:961: Vex Pro 1x1 rectangular tubing 2 in length:1 ↔ Hex Spacer:5
- Mate:962: Vex Pro 1x1 rectangular tubing 2 in length:1 ↔ Hex Spacer:5
- Mate:963: Hex Shaft 3-8 in (am-0855):1 ↔ Hex Spacer:5
- Mate:964: Vex Pro 1x1 rectangular tubing 2 in length:1 ↔ Hex Spacer:6
- Mate:965: Vex Pro 1x1 rectangular tubing 2 in length:1 ↔ Hex Spacer:6
- Mate:966: Hex Shaft 3-8 in (am-0855):1 ↔ Hex Spacer:6
- Mate:967: Vex Pro 1x1 rectangular tubing 2 in length:2 ↔ Hex Spacer:7
- Mate:968: Vex Pro 1x1 rectangular tubing 2 in length:2 ↔ Hex Spacer:7
- Mate:969: Hex Shaft 3-8 in (am-0855):1 ↔ Hex Spacer:7
- Mate:970: Vex Pro 1x1 rectangular tubing 2 in length:2 ↔ Hex Spacer:8
- Mate:971: Vex Pro 1x1 rectangular tubing 2 in length:2 ↔ Hex Spacer:8
- Mate:972: Hex Shaft 3-8 in (am-0855):1 ↔ Hex Spacer:8
- Mate:973: Vex Pro 1x1 rectangular tubing 14 in length:6 ↔ Bearing Mount Spacer 1-8 in:1
- Mate:974: Vex Pro 1x1 rectangular tubing 14 in length:6 ↔ Bearing Mount Spacer 1-8 in:3
- Mate:975: Vex Pro 1x1 rectangular tubing 14 in length:5 ↔ Bearing Mount Spacer 1-8 in:7
- Mate:976: Vex Pro 1x1 rectangular tubing 14 in length:6 ↔ Bearing Mount Spacer 1-8 in:1
- Mate:977: Vex Pro 1x1 rectangular tubing 14 in length:6 ↔ Vex Pro End Bearing Mount (Bolt):4
- Mate:978: Vex Pro 1x1 rectangular tubing 14 in length:6 ↔ Bearing Mount Spacer 1-8 in:3
- Mate:979: Vex Pro 1x1 rectangular tubing 14 in length:5 ↔ Vex Pro End Bearing Mount (Bolt):1
- Mate:980: Bearing Mount Spacer 1-8 in:7 ↔ Vex Pro End Bearing Mount (Bolt):1
- Mate:981: Vex Pro 1x1 rectangular tubing 14 in length:5 ↔ Vex Pro End Bearing Mount (Bolt):2
- Mate:983: Vex Pro 1x1 rectangular tubing 14 in length:5 ↔ Bearing Mount Spacer 1-8 in:5
- Mate:988: Vex Pro 1x1 rectangular tubing 14 in length (roller):1 ↔ Side Mount Custom:1
- Mate:989: Vex Pro 1x1 rectangular tubing 14 in length (roller):1 ↔ Side Mount Custom:1
- Mate:990: VersaPlanetary (Fixed):1 ↔ Side Mount Custom:1
- Mate:991: VersaPlanetary (Fixed):1 ↔ Side Mount Custom:1
- Mate:992: VersaPlanetary (Fixed):1 ↔ Side Mount Custom:1
- Mate:1020: Vex Pro 1x1 rectangular tubing 14 in length:6 ↔ Vex Pro 90 degree gusset:18
- Mate:1021: Vex Pro 1x1 rectangular tubing 14 in length:6 ↔ Vex Pro 90 degree gusset:18
- Mate:1022: Vex Pro 1x1 rectangular tubing 14 in length:5 ↔ Vex Pro 90 degree gusset:15
- Mate:1023: Vex Pro 1x1 rectangular tubing 14 in length:5 ↔ Vex Pro 90 degree gusset:15
- Mate:1024: Pneumatic Piston Back Flange (Right Custom):1 ↔ Clamp Piston ( 1 in stroke twice, 9-16 bore):1
- Mate:1025: Pneumatic Piston Back Flange (Right Custom):1 ↔ Clamp Piston ( 1 in stroke twice, 9-16 bore):1
- Mate:1026: Pneumatic Piston Back Flange (Right Custom):1 ↔ Clamp Piston ( 1 in stroke twice, 9-16 bore):1
- Mate:1028: Pneumatic Piston Back Flange (Rt Custom):1 ↔ Clamp Piston ( 1 in stroke twice, 9-16 bore):2
- Mate:1029: Pneumatic Piston Back Flange (Rt Custom):1 ↔ Clamp Piston ( 1 in stroke twice, 9-16 bore):2
- Mate:1030: Pneumatic Piston Back Flange (Rt Custom):1 ↔ Clamp Piston ( 1 in stroke twice, 9-16 bore):2
- Mate:1032: Hex Shaft 1-2 in 5 in long (am-0856):1 ↔ Hex Shaft Collar 1-2 in (7552K500):30
- Mate:1033: Hex Shaft 1-2 in 5 in long (am-0856):1 ↔ Hex Shaft Collar 1-2 in (7552K500):30
- Mate:1034: Gusset 3 (R-L) (Custom):1 ↔ Hex Shaft Collar 1-2 in (7552K500):30
- Mate:1038: Vex Pro 1x1 rectangular tubing 14 in length (roller):1 ↔ Hex Spacer 1-2 :1
- Mate:1039: Vex Pro 1x1 rectangular tubing 14 in length (roller):1 ↔ Hex Spacer 1-2 :1
- Mate:1040: Hex Shaft 1-2 in (am-0856):4 ↔ Hex Spacer 1-2 :1
- Mate:1041: Vex Pro 1x1 rectangular tubing 14 in length (roller):1 ↔ Hex Spacer 1-2 :2
- Mate:1042: Vex Pro 1x1 rectangular tubing 14 in length (roller):1 ↔ Hex Spacer 1-2 :2
- Mate:1043: Hex Shaft 1-2 in (am-0856):4 ↔ Hex Spacer 1-2 :2
- Mate:1044: Vex Pro 1x1 rectangular tubing 14 in length (roller):2 ↔ Hex Spacer 1-2 :3
- Mate:1045: Vex Pro 1x1 rectangular tubing 14 in length (roller):2 ↔ Hex Spacer 1-2 :3
- Mate:1046: Hex Shaft 1-2 in (am-0856):5 ↔ Hex Spacer 1-2 :3
- Mate:1047: Vex Pro 1x1 rectangular tubing 14 in length (roller):2 ↔ Hex Spacer 1-2 :4
- Mate:1048: Vex Pro 1x1 rectangular tubing 14 in length (roller):2 ↔ Hex Spacer 1-2 :4
- Mate:1049: Hex Shaft 1-2 in (am-0856):5 ↔ Hex Spacer 1-2 :4
- Flush:26: Vex Pro 1x1 rectangular tubing 14 in length:6 ↔ Vex Pro 1x1 rectangular tubing 14 in length (roller):1
- Mate:1050: Vex Pro 1x1 rectangular tubing 14 in length (roller):1 ↔ Side Mount Custom:1
- Flush:27: Vex Pro 1x1 rectangular tubing 14 in length:5 ↔ Vex Pro 1x1 rectangular tubing 14 in length (roller):2
- Mate:1053: Vex Pro 1x1 rectangular tubing 14 in length:5 ↔ Roller Piston 4 (.5 and 1 in Stroke, 9-16 in Bore):1
- Mate:1054: Vex Pro 1x1 rectangular tubing 14 in length:5 ↔ Roller Piston 4 (.5 and 1 in Stroke, 9-16 in Bore):1
- Mate:1055: Vex Pro 1x1 rectangular tubing 14 in length:5 ↔ Roller Piston 4 (.5 and 1 in Stroke, 9-16 in Bore):1
- Mate:1056: Vex Pro 1x1 rectangular tubing 14 in length:6 ↔ Roller Piston 4 (.5 and 1 in Stroke, 9-16 in Bore):2
- Mate:1057: Vex Pro 1x1 rectangular tubing 14 in length:6 ↔ Roller Piston 4 (.5 and 1 in Stroke, 9-16 in Bore):2
- Mate:1058: Vex Pro 1x1 rectangular tubing 14 in length:6 ↔ Roller Piston 4 (.5 and 1 in Stroke, 9-16 in Bore):2
- Mate:1059: Bracket:1 ↔ Roller Piston 4 (.5 and 1 in Stroke, 9-16 in Bore):2
- Mate:1060: Bracket:2 ↔ Roller Piston 4 (.5 and 1 in Stroke, 9-16 in Bore):1
- Mate:1061: Shaft Collar 3-16 in ID (6435K510):2 ↔ Roller Piston 4 (.5 and 1 in Stroke, 9-16 in Bore):1
- Mate:1062: Shaft Collar 3-16 in ID (6435K510):1 ↔ Roller Piston 4 (.5 and 1 in Stroke, 9-16 in Bore):1
- Mate:1063: Shaft Collar 3-16 in ID (6435K510):3 ↔ Roller Piston 4 (.5 and 1 in Stroke, 9-16 in Bore):2
- Mate:1064: Shaft Collar 3-16 in ID (6435K510):4 ↔ Roller Piston 4 (.5 and 1 in Stroke, 9-16 in Bore):2
- Mate:1065: Hex Shaft Aluminum 1-2 in (am-2291):1 ↔ Hex Shaft Collar 1-2 in (7552K500):31
- Mate:1066: Hex Shaft Aluminum 1-2 in (am-2291):1 ↔ Hex Shaft Collar 1-2 in (7552K500):31
- Mate:1067: Hex Bearing 1-2 in (FR8ZZ-Hex, am-0279):4 ↔ Hex Shaft Collar 1-2 in (7552K500):31
- Mate:1068: Hex Shaft Aluminum 1-2 in (am-2291):1 ↔ Timing Pulley (HTD 5mm) - 18T 9mm Double Flange, 1-2 in Hex (VexPro):5
- Mate:1069: Hex Shaft Aluminum 1-2 in (am-2291):1 ↔ Timing Pulley (HTD 5mm) - 18T 9mm Double Flange, 1-2 in Hex (VexPro):5
- Mate:1070: Hex Shaft Collar 1-2 in (7552K500):31 ↔ Timing Pulley (HTD 5mm) - 18T 9mm Double Flange, 1-2 in Hex (VexPro):5
- Mate:1071: Timing Pulley (HTD 5mm) - 18T 9mm Double Flange, 1-2 in Hex (VexPro):5 ↔ Hex Shaft Collar 1-2 in (7552K500):32
- Mate:1072: Hex Shaft Aluminum 1-2 in (am-2291):1 ↔ Hex Shaft Collar 1-2 in (7552K500):32
- Mate:1073: Hex Shaft Aluminum 1-2 in (am-2291):1 ↔ Hex Shaft Collar 1-2 in (7552K500):32
- [Mate]: Hex Shaft Collar 1-2 in (7552K500):33 ↔ Timing Pulley (HTD 5mm) - 18T 9mm Double Flange, 1-2 in Hex (VexPro):6
- [Mate]: Timing Pulley (HTD 5mm) - 18T 9mm Double Flange, 1-2 in Hex (VexPro):6 ↔ Hex Shaft Collar 1-2 in (7552K500):34
- Mate:1076: VersaPlanetary (Fixed):1 ↔ Hex Shaft Collar 1-2 in (7552K500):34
- Flush:29: Hex Shaft Collar 1-2 in (7552K500):32 ↔ Hex Shaft Collar 1-2 in (7552K500):34
- Mate:1077: VersaPlanetary (Fixed):1 ↔ Hex Shaft Collar 1-2 in (7552K500):34
- Mate:1078: Timing Pulley (HTD 5mm) - 18T 9mm Double Flange, 1-2 in Hex (VexPro):6 ↔ Hex Shaft Collar 1-2 in (7552K500):34
- Mate:1079: VersaPlanetary (Fixed):1 ↔ Timing Pulley (HTD 5mm) - 18T 9mm Double Flange, 1-2 in Hex (VexPro):6
- Mate:1080: VersaPlanetary (Fixed):1 ↔ Timing Pulley (HTD 5mm) - 18T 9mm Double Flange, 1-2 in Hex (VexPro):6
- Mate:1081: Hex Shaft Collar 1-2 in (7552K500):33 ↔ Timing Pulley (HTD 5mm) - 18T 9mm Double Flange, 1-2 in Hex (VexPro):6
- Mate:1082: VersaPlanetary (Fixed):1 ↔ Hex Shaft Collar 1-2 in (7552K500):33